# Autodesk Inventor assembly: arm j2 assemny
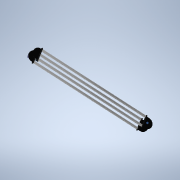
[picture p0: Inventor's stored thumbnail of the model, 180x180]
Saved by Autodesk Inventor 2020 (Build 240168000, 168)
## iProperties
Created: 2020-07-11
Part Number: arm j2 assemny
Document SubType Name: Assembly
Designer: Vikki
Mass: 15286.2 g
Surface Area: 29837.4 cm^2
Volume: 5661.55 cm^3
Density: 2.7 g/cm^3
Author: Vikki
## Documents named in this file (9)
- D:\projects\Intelligent Picking\vicky models\articulated arm\arm j2 assemny.iam
- D:\projects\Intelligent Picking\vicky models\articulated arm\arm j2.ipt
- D:\projects\Intelligent Picking\vicky models\articulated arm\2040ext 2200m.ipt
- D:\projects\Intelligent Picking\vicky models\articulated arm\arm j2 assemny\AIP\FEA\db2oahsww.fins
- D:\projects\Intelligent Picking\vicky models\articulated arm\arm j2 assemny\AIP\FEA\db2oahsww.fsat
- D:\projects\Intelligent Picking\vicky models\articulated arm\arm j2 assemny\AIP\FEA\db2oahsww.ftes
- D:\projects\Intelligent Picking\vicky models\articulated arm\arm j2 assemny\AIP\FEA\db2oahsww.fwiz
- D:\projects\Intelligent Picking\vicky models\articulated arm\arm j2 assemny\AIP\FEA\db2oahsxs.fmsh
- D:\projects\Intelligent Picking\vicky models\articulated arm\arm j2 assemny\AIP\FEA\db2oahsxt.fres
## Components (2 placed, 2 different names)
1. arm j2:1 — Mate:2, Mate:3, Flush:1, Flush:2, Flush:3
2. 2040ext 2200m:1 — Mate:2, Mate:3, Flush:1, Flush:2, Flush:3
## Relationships (5: Flush 3, Mate 2)
- Mate:2: arm j2:1 ↔ 2040ext 2200m:1
- Mate:3 (50 mm): arm j2:1 ↔ 2040ext 2200m:1
- Flush:1: arm j2:1 ↔ 2040ext 2200m:1
- Flush:2: arm j2:1 ↔ 2040ext 2200m:1
- Flush:3: arm j2:1 ↔ 2040ext 2200m:1
## Named parameters: sa_0 = 15000, sa_1 = 981
note: some values were not read from the file. Shown as the stored number, unit unknown: "sa_0", "sa_1".
